# Autodesk Inventor assembly: Eyes
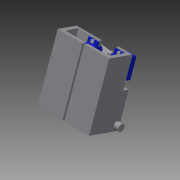
[picture p0: Inventor's stored thumbnail of the model, 180x180]
Saved by Autodesk Inventor 2013 (Build 170138000, 138)
## iProperties
Created: 2012-09-25
Part Number: Eyes
Document SubType Name: Assembly
Designer: uqgtayle
Author: uqgtayle
## Documents named in this file (19)
- G:\workshops-design\Mechanical\2012 Jobs\Grant\Animatronic Eyes\Eyes.iam
- G:\workshops-design\Mechanical\2012 Jobs\Grant\Animatronic Eyes\ping pong ball.ipt
- G:\workshops-design\Mechanical\2012 Jobs\Grant\Animatronic Eyes\Ball Ring.ipt
- G:\workshops-design\Mechanical\2012 Jobs\Grant\Animatronic Eyes\3mm Rod.ipt
- G:\workshops-design\Mechanical\2012 Jobs\Grant\Animatronic Eyes\5mm Screw.ipt
- G:\workshops-design\Mechanical\2012 Jobs\Grant\Animatronic Eyes\Right Angle.ipt
- G:\workshops-design\Mechanical\2012 Jobs\Grant\Animatronic Eyes\Left Angle.ipt
- G:\workshops-design\Mechanical\2012 Jobs\Grant\Animatronic Eyes\PVC Spacer.ipt
- G:\workshops-design\Mechanical\2012 Jobs\Grant\Animatronic Eyes\Servo Mount1.ipt
- G:\workshops-design\Mechanical\2012 Jobs\Grant\Animatronic Eyes\Servo Mount2.ipt
- G:\workshops-design\Mechanical\2012 Jobs\Grant\Animatronic Eyes\Servo Motor.ipt
- G:\workshops-design\Mechanical\2012 Jobs\Grant\Animatronic Eyes\Servo Arm.ipt
- G:\workshops-design\Mechanical\2012 Jobs\Grant\Animatronic Eyes\Link Arm1.ipt
- G:\workshops-design\Mechanical\2012 Jobs\Grant\Animatronic Eyes\Link Arm 2.ipt
- G:\workshops-design\Mechanical\2012 Jobs\Grant\Animatronic Eyes\Spring1.ipt
- G:\workshops-design\Mechanical\2012 Jobs\Grant\Animatronic Eyes\Spring2.ipt
- G:\workshops-design\Mechanical\2012 Jobs\Grant\Animatronic Eyes\M2 Screw.ipt
- G:\workshops-design\Mechanical\2012 Jobs\Grant\Animatronic Eyes\M2x6 Screw.ipt
- G:\workshops-design\Mechanical\2012 Jobs\Grant\Animatronic Eyes\M2 Nut.ipt
## Components (38 placed, 18 different names)
1. ping pong ball:1 — Mate:15, Tangent:2, Mate:39, Mate:72, Tangent:4
2. Ball Ring:1 — Mate:1, Mate:3, Mate:4, Mate:7, Mate:10, Mate:11, Mate:37, Mate:38, Tangent:1, Flush:2, Mate:40, Tangent:3, Mate:74
3. 3mm Rod:1 — Mate:1, Mate:13, Mate:14, Mate:15, Tangent:1
4. 5mm Screw:1 — Mate:3, Mate:8, Mate:9, Mate:10, Mate:11
5. 5mm Screw:2 — Mate:4, Mate:5, Mate:6, Mate:7
6. Right Angle:1 — Mate:5, Mate:6, Flush:1, Mate:20, Mate:21, Mate:22
7. Left Angle:1 — Mate:8, Mate:9, Flush:1, Mate:23, Mate:24, Mate:25
8. PVC Spacer:1 — Mate:14, Mate:38, Tangent:2
9. PVC Spacer:2 — Mate:13, Mate:37
10. Servo Mount1:1 — Mate:17, Mate:18, Mate:19, Mate:20, Mate:21, Mate:22, Mate:41, Mate:42, Mate:43, Mate:44, Mate:53, Mate:55
11. Servo Mount2:1 — Mate:23, Mate:24, Mate:25, Mate:26, Mate:27, Mate:28, Mate:45, Mate:46, Mate:47, Mate:48, Mate:51, Mate:57
12. Servo Motor:1 — Mate:26, Mate:27, Mate:28, Mate:31, Mate:32, Mate:52, Mate:58, Mate:63
13. Servo Motor:2 — Mate:17, Mate:18, Mate:19, Mate:29, Mate:30, Mate:54, Mate:56, Mate:61
14. Servo Arm:1 — Mate:29, Mate:30, Mate:35, Mate:49, Mate:50, Mate:62, Mate:66
15. Servo Arm:2 — Mate:31, Mate:32, Mate:33, Mate:34, Mate:59, Mate:60, Mate:64
16. Link Arm1:1 — Mate:35
17. Link Arm 2:1 — Mate:33, Mate:34, Mate:71
18. Spring1:1 — Mate:39
19. Spring2:1 — Mate:40, Tangent:3
20. M2 Screw:1 — Mate:41, Mate:42
21. M2 Screw:2 — Mate:43, Mate:44
22. M2 Screw:3 — Mate:49, Mate:50, Mate:65, Mate:67, Flush:3, Mate:68
23. M2 Screw:6 — Mate:45, Mate:46
24. M2 Screw:10 — Mate:47, Mate:48
25. M2x6 Screw:1 — Mate:51, Mate:52
26. M2x6 Screw:2 — Mate:57, Mate:58
27. M2x6 Screw:3 — Mate:59, Mate:60, Mate:70
28. M2x6 Screw:4 — Mate:55, Mate:56
29. M2x6 Screw:5 — Mate:53, Mate:54
30. M2x6 Screw:6 — Mate:61, Mate:62
31. M2x6 Screw:7 — Mate:63, Mate:64
32. M2 Nut:1 — Mate:68, Mate:69
33. M2 Nut:3 — Mate:73
34. M2 Nut:6 — Mate:67, Flush:3, Mate:69
35. M2 Nut:7 — Mate:65, Mate:66
36. M2 Nut:8 — Mate:70, Mate:71
37. M2x6 Screw:8 — Mate:72, Tangent:4, Mate:73
38. M2x6 Screw:9 — Mate:74
## Relationships (77: Mate 70, Tangent 4, Flush 3)
- Mate:1: Ball Ring:1 ↔ 3mm Rod:1
- Mate:3: Ball Ring:1 ↔ 5mm Screw:1
- Mate:4: Ball Ring:1 ↔ 5mm Screw:2
- Mate:5: 5mm Screw:2 ↔ Right Angle:1
- Mate:6: 5mm Screw:2 ↔ Right Angle:1
- Mate:7 (22 mm): Ball Ring:1 ↔ 5mm Screw:2
- Mate:8: 5mm Screw:1 ↔ Left Angle:1
- Mate:9: 5mm Screw:1 ↔ Left Angle:1
- Flush:1: Right Angle:1 ↔ Left Angle:1
- Mate:10: Ball Ring:1 ↔ 5mm Screw:1
- Mate:11 (22 mm): Ball Ring:1 ↔ 5mm Screw:1
- Mate:13: 3mm Rod:1 ↔ PVC Spacer:2
- Mate:14: 3mm Rod:1 ↔ PVC Spacer:1
- Mate:15: ping pong ball:1 ↔ 3mm Rod:1
- Mate:17: Servo Mount1:1 ↔ Servo Motor:2
- Mate:18: Servo Mount1:1 ↔ Servo Motor:2
- Mate:19: Servo Mount1:1 ↔ Servo Motor:2
- Mate:20: Right Angle:1 ↔ Servo Mount1:1
- Mate:21: Right Angle:1 ↔ Servo Mount1:1
- Mate:22: Right Angle:1 ↔ Servo Mount1:1
- Mate:23: Left Angle:1 ↔ Servo Mount2:1
- Mate:24: Left Angle:1 ↔ Servo Mount2:1
- Mate:25: Left Angle:1 ↔ Servo Mount2:1
- Mate:26: Servo Mount2:1 ↔ Servo Motor:1
- Mate:27: Servo Mount2:1 ↔ Servo Motor:1
- Mate:28: Servo Mount2:1 ↔ Servo Motor:1
- Mate:29: Servo Motor:2 ↔ Servo Arm:1
- Mate:30: Servo Motor:2 ↔ Servo Arm:1
- Mate:31: Servo Motor:1 ↔ Servo Arm:2
- Mate:32: Servo Motor:1 ↔ Servo Arm:2
- Mate:33: Servo Arm:2 ↔ Link Arm 2:1
- Mate:34 (2 mm): Servo Arm:2 ↔ Link Arm 2:1
- Mate:35: Servo Arm:1 ↔ Link Arm1:1
- Mate:37: Ball Ring:1 ↔ PVC Spacer:2
- Mate:38: Ball Ring:1 ↔ PVC Spacer:1
- Tangent:1 (-58 mm): Ball Ring:1 ↔ 3mm Rod:1
- Tangent:2: ping pong ball:1 ↔ PVC Spacer:1
- Mate:39: ping pong ball:1 ↔ Spring1:1
- Flush:2: Ball Ring:1
- Mate:40: Ball Ring:1 ↔ Spring2:1
- Tangent:3: Ball Ring:1 ↔ Spring2:1
- Mate:41: Servo Mount1:1 ↔ M2 Screw:1
- Mate:42: Servo Mount1:1 ↔ M2 Screw:1
- Mate:43: Servo Mount1:1 ↔ M2 Screw:2
- Mate:44: Servo Mount1:1 ↔ M2 Screw:2
- Mate:45: Servo Mount2:1 ↔ M2 Screw:6
- Mate:46: Servo Mount2:1 ↔ M2 Screw:6
- Mate:47: Servo Mount2:1 ↔ M2 Screw:10
- Mate:48: Servo Mount2:1 ↔ M2 Screw:10
- Mate:49: Servo Arm:1 ↔ M2 Screw:3
- Mate:50: Servo Arm:1 ↔ M2 Screw:3
- Mate:51: Servo Mount2:1 ↔ M2x6 Screw:1
- Mate:52: Servo Motor:1 ↔ M2x6 Screw:1
- Mate:53: Servo Mount1:1 ↔ M2x6 Screw:5
- Mate:54: Servo Motor:2 ↔ M2x6 Screw:5
- Mate:55: Servo Mount1:1 ↔ M2x6 Screw:4
- Mate:56: Servo Motor:2 ↔ M2x6 Screw:4
- Mate:57: Servo Mount2:1 ↔ M2x6 Screw:2
- Mate:58: Servo Motor:1 ↔ M2x6 Screw:2
- Mate:59: Servo Arm:2 ↔ M2x6 Screw:3
- Mate:60: Servo Arm:2 ↔ M2x6 Screw:3
- Mate:61: Servo Motor:2 ↔ M2x6 Screw:6
- Mate:62: Servo Arm:1 ↔ M2x6 Screw:6
- Mate:63: Servo Motor:1 ↔ M2x6 Screw:7
- Mate:64: Servo Arm:2 ↔ M2x6 Screw:7
- Mate:65: M2 Screw:3 ↔ M2 Nut:7
- Mate:66: Servo Arm:1 ↔ M2 Nut:7
- Mate:67: M2 Screw:3 ↔ M2 Nut:6
- Flush:3: M2 Screw:3 ↔ M2 Nut:6
- Mate:68: M2 Screw:3 ↔ M2 Nut:1
- Mate:69: M2 Nut:1 ↔ M2 Nut:6
- Mate:70: M2x6 Screw:3 ↔ M2 Nut:8
- Mate:71: Link Arm 2:1 ↔ M2 Nut:8
- Mate:72: ping pong ball:1 ↔ M2x6 Screw:8
- Tangent:4: ping pong ball:1 ↔ M2x6 Screw:8
- Mate:73: M2 Nut:3 ↔ M2x6 Screw:8
- Mate:74: Ball Ring:1 ↔ M2x6 Screw:9
